# Autodesk Inventor assembly: POM_T5_14
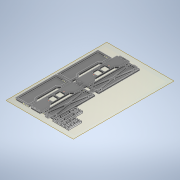
[picture p0: Inventor's stored thumbnail of the model, 180x180]
Saved by Autodesk Inventor 2022 (Build 260153000, 153)
## iProperties
Created: 2022-09-28
Part Number: POM_T5_14
Document SubType Name: Assembly
Designer: Masato
Author: Masato
## Documents named in this file (7)
- C:\Users\ヨコオリク\Documents\CITBrains\SUSTAINA-OP\Cam\POM_T5\POM_T5_14.iam
- C:\Users\ヨコオリク\Documents\CITBrains\SUSTAINA-OP\Cam\DisposableBoard.ipt
- C:\Users\ヨコオリク\Documents\CITBrains\SUSTAINA-OP\UpperBody\Cockpit\Cockpit_battery_frame.ipt
- C:\Users\ヨコオリク\Documents\CITBrains\SUSTAINA-OP\UpperBody\Cockpit\Cockpit_top_frame.ipt
- C:\Users\ヨコオリク\Documents\CITBrains\SUSTAINA-OP\OptionParts\DrillingJigs\Cockpit_back_frame_Jig.ipt
- C:\Users\ヨコオリク\Documents\CITBrains\SUSTAINA-OP\OptionParts\DrillingJigs\Cockpit_battery_frame_Jig.ipt
- C:\Users\ヨコオリク\Documents\CITBrains\SUSTAINA-OP\UpperBody\Cockpit\Cockpit_battery_back_door.ipt
## Components (11 placed, 6 different names)
1. DisposableBoard:1 — フラッシュ:1, フラッシュ:2, フラッシュ:3, フラッシュ:4, フラッシュ:12, フラッシュ:13, フラッシュ:14, フラッシュ:15, フラッシュ:16
2. Cockpit_battery_back_door:1 — メイト:48, フラッシュ:13, フラッシュ:14, メイト:49
3. Cockpit_battery_back_door:2
4. Cockpit_top_frame:1 — メイト:8, フラッシュ:7, メイト:13, メイト:49, フラッシュ:15
5. Cockpit_top_frame:3
6. Cockpit_battery_frame:1 — メイト:4, フラッシュ:7, メイト:13, メイト:33
7. Cockpit_battery_frame:3
8. Cockpit_back_frame_Jig:1 — メイト:32, フラッシュ:12, メイト:33
9. Cockpit_back_frame_Jig:2 — メイト:50
10. Cockpit_battery_frame_Jig:1 — メイト:21, メイト:50, フラッシュ:16
11. Cockpit_battery_frame_Jig:3
## Component patterns: (2 elements, first: Cockpit_battery_back_door:1), (2 elements, first: Cockpit_top_frame:1), (2 elements, first: Cockpit_battery_frame:1), (2 elements, first: Cockpit_back_frame_Jig:1), (2 elements, first: Cockpit_battery_frame_Jig:1)
## Relationships (19: Flush 10, Mate 9)
- フラッシュ:1 [Flush]: DisposableBoard:1
- フラッシュ:2 [Flush]: DisposableBoard:1
- フラッシュ:3 [Flush]: DisposableBoard:1
- フラッシュ:4 [Flush]: DisposableBoard:1
- メイト:4 [Mate]: Cockpit_battery_frame:1
- メイト:8 [Mate]: Cockpit_top_frame:1
- フラッシュ:7 [Flush]: Cockpit_top_frame:1 ↔ Cockpit_battery_frame:1
- メイト:13 [Mate] (2.1 mm): Cockpit_top_frame:1 ↔ Cockpit_battery_frame:1
- メイト:21 [Mate]: Cockpit_battery_frame_Jig:1
- メイト:32 [Mate]: Cockpit_back_frame_Jig:1
- フラッシュ:12 [Flush] (2 mm): DisposableBoard:1 ↔ Cockpit_back_frame_Jig:1
- メイト:33 [Mate] (2.1 mm): Cockpit_battery_frame:1 ↔ Cockpit_back_frame_Jig:1
- メイト:48 [Mate]: Cockpit_battery_back_door:1
- フラッシュ:13 [Flush] (2 mm): DisposableBoard:1 ↔ Cockpit_battery_back_door:1
- フラッシュ:14 [Flush] (2 mm): DisposableBoard:1 ↔ Cockpit_battery_back_door:1
- メイト:49 [Mate] (2.1 mm): Cockpit_battery_back_door:1 ↔ Cockpit_top_frame:1
- フラッシュ:15 [Flush] (2 mm): DisposableBoard:1 ↔ Cockpit_top_frame:1
- メイト:50 [Mate] (2.1 mm): Cockpit_back_frame_Jig:2 ↔ Cockpit_battery_frame_Jig:1
- フラッシュ:16 [Flush] (2 mm): DisposableBoard:1 ↔ Cockpit_battery_frame_Jig:1
